# Autodesk Inventor assembly: BAG_2_3-8inHex
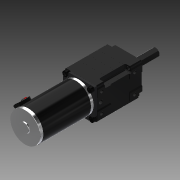
[picture p0: Inventor's stored thumbnail of the model, 180x180]
Saved by Autodesk Inventor 2022 (Build 260153000, 153)
## iProperties
Created: 2018-08-19
Part Number: BAG_2_3-8inHex
Document SubType Name: Assembly
Mass: 1123.04 g
Surface Area: 1203.25 cm^2
Volume: 285.054 cm^3
Density: 3.93975 g/cm^3
## Documents named in this file (10)
- E:\Middleton Robotics\Collaborative Robots\Collaborative Part Library\General Gearboxes\Planetaries\Versaplanetary\VersaPlanetary\BAG, 2 Stages, 3-8in Hex Output.iam
- E:\Middleton Robotics\Collaborative Robots\Collaborative Part Library\General Gearboxes\Planetaries\Versaplanetary\V2 Stages\V2 Output Stage.iam
- E:\Middleton Robotics\Collaborative Robots\Collaborative Part Library\General Gearboxes\Planetaries\Versaplanetary\Intermediate Stages\Ring Gear.ipt
- E:\Middleton Robotics\Collaborative Robots\Collaborative Part Library\General Gearboxes\Planetaries\Versaplanetary\V2 Stages\V2 Input Stage.iam
- E:\Middleton Robotics\Collaborative Robots\Collaborative Part Library\General Gearboxes\Planetaries\Versaplanetary\Screws\8-32 x 2.25in Screw.ipt
- E:\Middleton Robotics\Collaborative Robots\Collaborative Part Library\Power Transfer\Bearings and Bushings\Bearings\6902ZZ.ipt
- E:\Middleton Robotics\Collaborative Robots\Collaborative Part Library\Power Transfer\Bearings.ipt
- E:\Middleton Robotics\Collaborative Robots\Collaborative Part Library\General Gearboxes\Planetaries\Versaplanetary\VersaPlanetary.iam
- E:\Middleton Robotics\Collaborative Robots\Collaborative Part Library\General Gearboxes\Planetaries\Versaplanetary\V2 Stages\V2 Output Stage\VP V2 Output Stage 3-8in Hex.iam
- E:\Middleton Robotics\Collaborative Robots\Collaborative Part Library\General Gearboxes\Planetaries\Versaplanetary\V2 Stages\V2 Input Stage\VP BAG Input.iam
## Components (8 placed, 6 different names)
1. VP V2 Output Stage 3-8in Hex:3 [sub-assembly] — Insert:1, Flush:3, Flush:6, 2StageBasicInputMate2, Insert:25
2. Ring Gear 1 — Insert:1, Insert:2, Flush:1, Flush:3
3. Ring Gear 2 — Insert:2, Flush:1, Flush:6, 2StageBasicInputMate1
4. VP BAG Input:1 [sub-assembly] — 2StageBasicInputMate1, 2StageBasicInputMate2, Insert:10, Insert:11
5. 8-32 x 2.25in Screw:1 — Insert:10
6. 8-32 x 2.25in Screw:2 — Insert:11
7. 6902ZZ:1
8. 6902ZZ:2 — Insert:25
## Relationships (10: Insert 6, Flush 4)
- Insert:1: VP V2 Output Stage 3-8in Hex:3 ↔ Ring Gear 1
- Insert:2: Ring Gear 1 ↔ Ring Gear 2
- Flush:1: Ring Gear 1 ↔ Ring Gear 2
- Flush:3: VP V2 Output Stage 3-8in Hex:3 ↔ Ring Gear 1
- Flush:6: VP V2 Output Stage 3-8in Hex:3 ↔ Ring Gear 2
- 2StageBasicInputMate1 [Insert]: Ring Gear 2 ↔ VP BAG Input:1
- 2StageBasicInputMate2 [Flush]: VP V2 Output Stage 3-8in Hex:3 ↔ VP BAG Input:1
- Insert:10: VP BAG Input:1 ↔ 8-32 x 2.25in Screw:1
- Insert:11: VP BAG Input:1 ↔ 8-32 x 2.25in Screw:2
- Insert:25: VP V2 Output Stage 3-8in Hex:3 ↔ 6902ZZ:2
